# Autodesk Inventor assembly: elevator
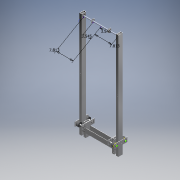
[picture p0: Inventor's stored thumbnail of the model, 180x180]
Saved by Autodesk Inventor 2017 (Build 210142000, 142)
## iProperties
Created: 2017-12-27
Part Number: elevator
Document SubType Name: Assembly
Designer: Micah
Mass: 4635.04 g
Surface Area: 10973.2 cm^2
Volume: 1751.48 cm^3
Density: 2.64636 g/cm^3
Author: Micah
## Documents named in this file (7)
- C:\Users\Micah\Desktop\inventor\CADathon-2017\2AM-17-A-0200 - Smokestack Elevator\2AM-17-A-0200 - elevator.iam
- C:\Users\Micah\Desktop\inventor\CADathon-2017\2AM-17-A-0200 - Smokestack Elevator\2AM-17-P-0201 - main structure.ipt
- C:\Users\Micah\Desktop\inventor\CADathon-2017\2AM-17-A-0200 - Smokestack Elevator\COTS\0_500_Hex_ID_x_1_125_OD_x_0_313_WD_Flanged_Bearing_v2_217-3875.ipt
- C:\Users\Micah\Desktop\inventor\CADathon-2017\2AM-17-A-0200 - Smokestack Elevator\2AM-17-P-0204 - top hex shaft.ipt
- C:\Users\Micah\Desktop\inventor\CADathon-2017\2AM-17-A-0200 - Smokestack Elevator\COTS\217-2737.20121205.ipt
- C:\Users\Micah\Desktop\inventor\CADathon-2017\2AM-17-A-0200 - Smokestack Elevator\COTS\_22t_Aluminum_Hub_Sprocket_25_Chain_1_2_Hex_Bore_217-2640.ipt
- C:\Users\Micah\Desktop\inventor\CADathon-2017\2AM-17-A-0200 - Smokestack Elevator\2AM-17-A-1200 - moving part.iam
## Components (10 placed, 6 different names)
1. 2AM-17-P-0201 - main structure:2 — Mate:4, Mate:6
2. 2AM-17-P-0201 - main structure:3 — Mate:5, Mate:7
3. 0_500_Hex_ID_x_1_125_OD_x_0_313_WD_Flanged_Bearing_v2_217-3875:1 — Mate:4, Rigid:1
4. 0_500_Hex_ID_x_1_125_OD_x_0_313_WD_Flanged_Bearing_v2_217-3875:2 — Mate:5
5. 2AM-17-P-0204 - top hex shaft:1 — Rigid:1, Rigid:2, Rigid:3
6. 217-2737.20121205:1 — Rigid:2, Insert:1
7. 217-2737.20121205:2 — Rigid:3, Insert:2
8. _22t_Aluminum_Hub_Sprocket_25_Chain_1_2_Hex_Bore_217-2640:1 — Insert:1
9. _22t_Aluminum_Hub_Sprocket_25_Chain_1_2_Hex_Bore_217-2640:2 — Insert:2
10. 2AM-17-A-1200 - moving part:1 [sub-assembly] — Mate:6, Mate:7
## Relationships (9: Mate 4, WeldJoint 3, Insert 2)
- Mate:4: 2AM-17-P-0201 - main structure:2 ↔ 0_500_Hex_ID_x_1_125_OD_x_0_313_WD_Flanged_Bearing_v2_217-3875:1
- Mate:5: 2AM-17-P-0201 - main structure:3 ↔ 0_500_Hex_ID_x_1_125_OD_x_0_313_WD_Flanged_Bearing_v2_217-3875:2
- Rigid:1 [WeldJoint] (-14.2875 mm): 0_500_Hex_ID_x_1_125_OD_x_0_313_WD_Flanged_Bearing_v2_217-3875:1 ↔ 2AM-17-P-0204 - top hex shaft:1
- Rigid:2 [WeldJoint]: 2AM-17-P-0204 - top hex shaft:1 ↔ 217-2737.20121205:1
- Rigid:3 [WeldJoint]: 2AM-17-P-0204 - top hex shaft:1 ↔ 217-2737.20121205:2
- Insert:1 (115.443 mm): 217-2737.20121205:1 ↔ _22t_Aluminum_Hub_Sprocket_25_Chain_1_2_Hex_Bore_217-2640:1
- Insert:2 (115.443 mm): 217-2737.20121205:2 ↔ _22t_Aluminum_Hub_Sprocket_25_Chain_1_2_Hex_Bore_217-2640:2
- Mate:6: 2AM-17-P-0201 - main structure:2 ↔ 2AM-17-A-1200 - moving part:1
- Mate:7: 2AM-17-P-0201 - main structure:3 ↔ 2AM-17-A-1200 - moving part:1
